# Autodesk Inventor assembly: Shoulder
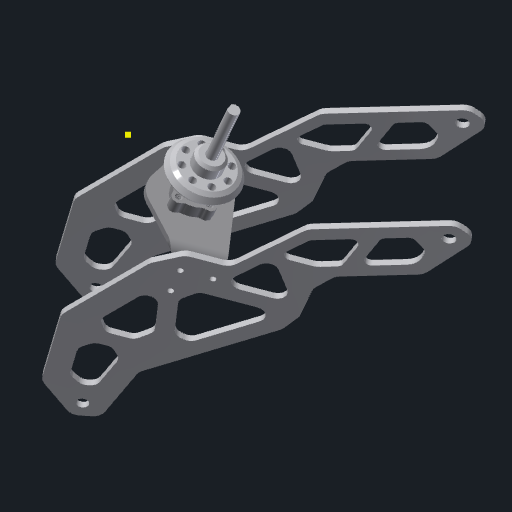
[picture p0: Inventor's stored thumbnail of the model, 512x512]
Saved by Autodesk Inventor 2023 (Build 270158000, 158)
## iProperties
Created: 2020-03-24
Part Number: Shoulder
Document SubType Name: Assembly
Designer: valer
Mass: 4853.13 g
Surface Area: 3141.52 cm^2
Volume: 1403.99 cm^3
Density: 3.45667 g/cm^3
Author: valer
## Documents named in this file (7)
- C:\Users\valer\Desktop\str1ker\cad\Shoulder.iam
- C:\Users\valer\Desktop\str1ker\cad\UpperArmBracket.ipt
- C:\Users\valer\Desktop\str1ker\cad\external\ShoulderMiterGear.ipt
- C:\Users\valer\Desktop\str1ker\cad\external\ShoulderShaft.ipt
- C:\Users\valer\Desktop\str1ker\cad\external\Shoulder6mmDShaftHub-545578.ipt
- C:\Users\valer\Desktop\str1ker\cad\UpperArmBracketBase.ipt
- C:\Users\valer\Desktop\str1ker\cad\ShoulderBoundingBox.ipt
## Components (7 placed, 6 different names)
1. UpperArmBracket:5 — Mate:386, Mate:387, Mate:392, Angle:1, Angle:3
2. UpperArmBracket:6 — Mate:384, Mate:385, Mate:391
3. ShoulderMiterGear:2 — Mate:382, Mate:389
4. ShoulderServoShaft:2 — Mate:374, Mate:382, Flush:1, Mate:383
5. Shoulder6mmDShaftHub-545578:1 — Mate:374, Flush:1, Mate:388, Mate:389, Mate:390
6. UpperArmBracketBase:1 — Mate:383, Mate:384, Mate:385, Mate:386, Mate:387, Mate:388, Mate:391, Mate:392, Angle:2, Angle:4
7. ShoulderBoundingBox:1 — Mate:393, Angle:3, Angle:4
## Relationships (18: Mate 13, Angle 4, Flush 1)
- Mate:374: ShoulderServoShaft:2 ↔ Shoulder6mmDShaftHub-545578:1
- Mate:382: ShoulderMiterGear:2 ↔ ShoulderServoShaft:2
- Flush:1 (-4 mm): ShoulderServoShaft:2 ↔ Shoulder6mmDShaftHub-545578:1
- Mate:383: ShoulderServoShaft:2 ↔ UpperArmBracketBase:1
- Mate:384: UpperArmBracket:6 ↔ UpperArmBracketBase:1
- Mate:385: UpperArmBracket:6 ↔ UpperArmBracketBase:1
- Mate:386: UpperArmBracket:5 ↔ UpperArmBracketBase:1
- Mate:387: UpperArmBracket:5 ↔ UpperArmBracketBase:1
- Mate:388: Shoulder6mmDShaftHub-545578:1 ↔ UpperArmBracketBase:1
- Mate:389 (10.9982 mm): ShoulderMiterGear:2 ↔ Shoulder6mmDShaftHub-545578:1
- Mate:390: Shoulder6mmDShaftHub-545578:1
- Mate:391: UpperArmBracket:6 ↔ UpperArmBracketBase:1
- Mate:392: UpperArmBracket:5 ↔ UpperArmBracketBase:1
- Angle:1 (0 deg): UpperArmBracket:5
- Angle:2 (0 deg): UpperArmBracketBase:1
- Mate:393: ShoulderBoundingBox:1
- Angle:3 (0 deg): UpperArmBracket:5 ↔ ShoulderBoundingBox:1
- Angle:4 (0 deg): UpperArmBracketBase:1 ↔ ShoulderBoundingBox:1
